# Autodesk Inventor assembly: Mold Assembly
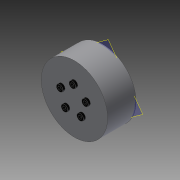
[picture p0: Inventor's stored thumbnail of the model, 180x180]
Saved by Autodesk Inventor 2013 (Build 170138000, 138)
## iProperties
Created: 2013-05-10
Part Number: Mold Assembly
Document SubType Name: Assembly
Designer: grtstudent
Author: grtstudent
## Documents named in this file (5)
- Z:\GRT 2013 Students\Rauhul Varma\Post Comp wheel tests\mold tests\Mold Assembly.iam
- Z:\GRT 2013 Students\Rauhul Varma\Post Comp wheel tests\mold tests\Aluminum mold support.ipt
- Z:\GRT 2013 Students\Rauhul Varma\Post Comp wheel tests\mold tests\moldmaybe.ipt
- Z:\GRT 2013 Students\Rauhul Varma\Post Comp wheel tests\mold tests\6-32 nylock.ipt
- Z:\GRT 2013 Students\Rauhul Varma\Post Comp wheel tests\mold tests\Rod Nut Side.ipt
## Components (12 placed, 4 different names)
1. Aluminum mold support:1 — Mate:1, Mate:2, Mate:3, Insert:1, Insert:2, Insert:3, Insert:4, Insert:5
2. moldmaybe:1 — Mate:1, Mate:2, Mate:3, Mate:4, Mate:5, Mate:6, Mate:7, Mate:8, Flush:5
3. 6-32 nylock:1 — Mate:5, Flush:1, Flush:5
4. 6-32 nylock:2 — Mate:4, Flush:3
5. 6-32 nylock:3 — Mate:6, Flush:2, Flush:3, Flush:4
6. 6-32 nylock:4 — Mate:7, Flush:1, Flush:2
7. 6-32 nylock:5 — Mate:8, Flush:4
8. Rod Nut Side:1 — Flush:6, Insert:1
9. Rod Nut Side:2 — Flush:6, Flush:7, Flush:8, Insert:2
10. Rod Nut Side:3 — Flush:8, Flush:9, Insert:4
11. Rod Nut Side:4 — Flush:9, Insert:5
12. Rod Nut Side:5 — Flush:7, Insert:3
## Relationships (22: Flush 9, Mate 8, Insert 5)
- Mate:1: Aluminum mold support:1 ↔ moldmaybe:1
- Mate:2: Aluminum mold support:1 ↔ moldmaybe:1
- Mate:3: Aluminum mold support:1 ↔ moldmaybe:1
- Mate:4: moldmaybe:1 ↔ 6-32 nylock:2
- Mate:5: moldmaybe:1 ↔ 6-32 nylock:1
- Mate:6: moldmaybe:1 ↔ 6-32 nylock:3
- Mate:7: moldmaybe:1 ↔ 6-32 nylock:4
- Mate:8: moldmaybe:1 ↔ 6-32 nylock:5
- Flush:1: 6-32 nylock:1 ↔ 6-32 nylock:4
- Flush:2: 6-32 nylock:3 ↔ 6-32 nylock:4
- Flush:3: 6-32 nylock:2 ↔ 6-32 nylock:3
- Flush:4: 6-32 nylock:3 ↔ 6-32 nylock:5
- Flush:5 (2.3813 mm): moldmaybe:1 ↔ 6-32 nylock:1
- Flush:6: Rod Nut Side:1 ↔ Rod Nut Side:2
- Flush:7: Rod Nut Side:2 ↔ Rod Nut Side:5
- Flush:8: Rod Nut Side:2 ↔ Rod Nut Side:3
- Flush:9: Rod Nut Side:3 ↔ Rod Nut Side:4
- Insert:1: Aluminum mold support:1 ↔ Rod Nut Side:1
- Insert:2: Aluminum mold support:1 ↔ Rod Nut Side:2
- Insert:3: Aluminum mold support:1 ↔ Rod Nut Side:5
- Insert:4: Aluminum mold support:1 ↔ Rod Nut Side:3
- Insert:5: Aluminum mold support:1 ↔ Rod Nut Side:4
